# Autodesk Inventor assembly: typea-x-assembly
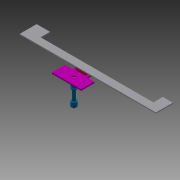
[picture p0: Inventor's stored thumbnail of the model, 180x180]
Saved by Autodesk Inventor 2014 (Build 180170000, 170)
## iProperties
Created: 2014-11-01
Part Number: typea-x-assembly
Document SubType Name: Assembly
Designer: caleb
Author: caleb
## Documents named in this file (5)
- C:\cygwin\home\caleb\caleb-typea-settings\designs\bowden-extruder\typea-x-assembly.iam
- C:\cygwin\home\caleb\caleb-typea-settings\designs\bowden-extruder\typea-x-rail.ipt
- C:\cygwin\home\caleb\caleb-typea-settings\designs\bowden-extruder\linear rail.ipt
- C:\cygwin\home\caleb\caleb-typea-settings\designs\bowden-extruder\linear slide.ipt
- C:\cygwin\home\caleb\caleb-typea-settings\designs\bowden-extruder\hotend carrier.ipt
## Components (4 placed, 4 different names)
1. typea-x-rail:1 — Mate:1, Flush:1
2. linear rail:1 — Mate:1, Flush:1, Mate:2, Mate:3
3. linear slide:1 — Mate:2, Mate:3, Mate:4, Mate:5, Mate:6
4. hotend carrier:1 — Mate:4, Mate:5, Mate:6
## Relationships (7: Mate 6, Flush 1)
- Mate:1: typea-x-rail:1 ↔ linear rail:1
- Flush:1 (-9.1 mm): typea-x-rail:1 ↔ linear rail:1
- Mate:2: linear rail:1 ↔ linear slide:1
- Mate:3: linear rail:1 ↔ linear slide:1
- Mate:4: linear slide:1 ↔ hotend carrier:1
- Mate:5: linear slide:1 ↔ hotend carrier:1
- Mate:6: linear slide:1 ↔ hotend carrier:1
